# Autodesk Inventor assembly: IGUS Drag Chain
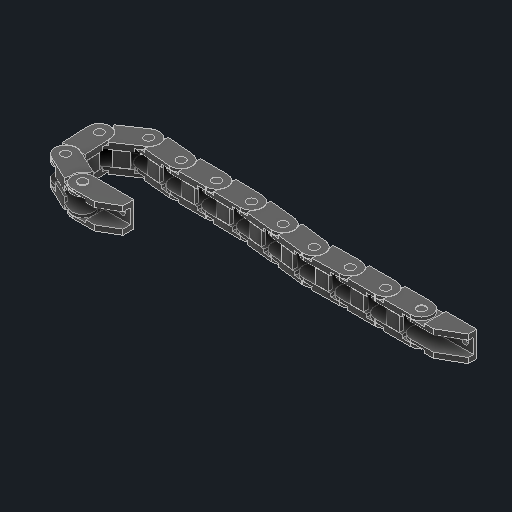
[picture p0: Inventor's stored thumbnail of the model, 512x512]
Saved by Autodesk Inventor 2025.1 (Build 291241020, 241B)
## iProperties
Created: 2025-05-09
Part Number: IGUS Drag Chain
Document SubType Name: Assembly
Designer: AdminForWorker
Title: IGUS Drag Chain
Author: AdminForWorker
## Documents named in this file (4)
- C:\Users\Joshua Eah\Documents\Voron 0.2\CAD\Master Assembly\IGUS Drag Chain.iam
- C:\Users\Joshua Eah\Documents\Voron 0.2\CAD\Master Assembly\E04-07-015-0 (7x7).ipt
- C:\Users\Joshua Eah\Documents\Voron 0.2\CAD\Master Assembly\040-07-12.ipt
- C:\Users\Joshua Eah\Documents\Voron 0.2\CAD\Master Assembly\040-07-12 (1).ipt
## Components (13 placed, 3 different names)
1. E04-07-015-0 (7x7):1 — Mate:2, Flush:2, Mate:3, Flush:3
2. 040-07-12:1 — Mate:12, Flush:12
3. 040-07-12 (1):1 — Mate:1, Flush:1
4. E04-07-015-0 (7x7):2 — Mate:3, Flush:3, Mate:4, Flush:4
5. E04-07-015-0 (7x7):3 — Mate:1, Mate:2, Flush:1, Flush:2
6. E04-07-015-0 (7x7):4 — Mate:6, Flush:6, Mate:7, Flush:7
7. E04-07-015-0 (7x7):5 — Mate:4, Flush:4, Mate:5, Flush:5
8. E04-07-015-0 (7x7):6 — Mate:10, Flush:10, Mate:11, Flush:11
9. E04-07-015-0 (7x7):7 — Mate:9, Flush:9, Mate:10, Flush:10
10. E04-07-015-0 (7x7):8 — Mate:8, Flush:8, Mate:9, Flush:9
11. E04-07-015-0 (7x7):9 — Mate:7, Flush:7, Mate:8, Flush:8
12. E04-07-015-0 (7x7):10 — Mate:5, Flush:5, Mate:6, Flush:6
13. E04-07-015-0 (7x7):11 — Mate:11, Flush:11, Mate:12, Flush:12
## Relationships (24: Mate 12, Flush 12)
- Mate:1: 040-07-12 (1):1 ↔ E04-07-015-0 (7x7):3
- Mate:2: E04-07-015-0 (7x7):1 ↔ E04-07-015-0 (7x7):3
- Flush:1: 040-07-12 (1):1 ↔ E04-07-015-0 (7x7):3
- Flush:2: E04-07-015-0 (7x7):1 ↔ E04-07-015-0 (7x7):3
- Mate:3: E04-07-015-0 (7x7):1 ↔ E04-07-015-0 (7x7):2
- Flush:3: E04-07-015-0 (7x7):1 ↔ E04-07-015-0 (7x7):2
- Mate:4: E04-07-015-0 (7x7):2 ↔ E04-07-015-0 (7x7):5
- Flush:4: E04-07-015-0 (7x7):2 ↔ E04-07-015-0 (7x7):5
- Mate:5: E04-07-015-0 (7x7):5 ↔ E04-07-015-0 (7x7):10
- Flush:5: E04-07-015-0 (7x7):5 ↔ E04-07-015-0 (7x7):10
- Mate:6: E04-07-015-0 (7x7):4 ↔ E04-07-015-0 (7x7):10
- Flush:6: E04-07-015-0 (7x7):4 ↔ E04-07-015-0 (7x7):10
- Mate:7: E04-07-015-0 (7x7):4 ↔ E04-07-015-0 (7x7):9
- Flush:7: E04-07-015-0 (7x7):4 ↔ E04-07-015-0 (7x7):9
- Mate:8: E04-07-015-0 (7x7):8 ↔ E04-07-015-0 (7x7):9
- Flush:8: E04-07-015-0 (7x7):8 ↔ E04-07-015-0 (7x7):9
- Mate:9: E04-07-015-0 (7x7):7 ↔ E04-07-015-0 (7x7):8
- Flush:9: E04-07-015-0 (7x7):7 ↔ E04-07-015-0 (7x7):8
- Mate:10: E04-07-015-0 (7x7):6 ↔ E04-07-015-0 (7x7):7
- Flush:10: E04-07-015-0 (7x7):6 ↔ E04-07-015-0 (7x7):7
- Mate:11: E04-07-015-0 (7x7):6 ↔ E04-07-015-0 (7x7):11
- Flush:11: E04-07-015-0 (7x7):6 ↔ E04-07-015-0 (7x7):11
- Mate:12: 040-07-12:1 ↔ E04-07-015-0 (7x7):11
- Flush:12: 040-07-12:1 ↔ E04-07-015-0 (7x7):11
